# Autodesk Inventor assembly: SimplifiedLeg040x
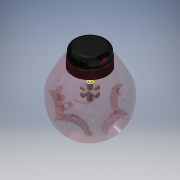
[picture p0: Inventor's stored thumbnail of the model, 180x180]
Saved by Autodesk Inventor 2018 (Build 220112000, 112)
## iProperties
Part Number: SimplifiedLeg040x
Material: Generisch
Document SubType Name: Assembly
Designer: Jochen Alt
Mass: 279.988 g
Surface Area: 1394.51 cm^2
Volume: 279.988 cm^3
Density: 1 g/cm^3
Author: Jochen Alt
## Documents named in this file (9)
- D:\Projects\Manfred\design\cad\simplified\SimplifiedLeg040x.iam
- D:\Projects\Manfred\design\cad\simplified\DrehAchse.ipt
- D:\Projects\Manfred\design\cad\simplified\SimplifiedFoot040x.ipt
- D:\Projects\Manfred\design\cad\simplified\SimplifiedThigh040x.ipt
- D:\Projects\Manfred\design\cad\simplified\SimplifiedHipJoint040x.ipt
- D:\Projects\Manfred\design\cad\simplified\SimplifiedHip040x.ipt
- D:\Projects\Manfred\design\cad\simplified\SimplifiedKnee040x.ipt
- D:\Projects\Manfred\design\cad\simplified\SimplifiedBody040x.ipt
- D:\Projects\Manfred\design\cad\Inventor\RPLidar A2.ipt
## Components (8 placed, 8 different names)
1. DrehAchse:1 — Passend:6, Passend:7, Passend:8, Passend:9, Passend:10, Passend:11, Passend:13, Passend:14, Winkel:1, Passend:15, Winkel:2
2. SimplifiedFoot040x:1 — Passend:6
3. SimplifiedThigh040x:1 — Passend:7, Passend:8
4. SimplifiedHipJoint040x:1 — Passend:9, Passend:10
5. SimplifiedHip040x:1 — Passend:11, Passend:15
6. SimplifiedKnee040x:1 — Passend:13, Passend:14, Winkel:1
7. SimplifiedBody040x:1 — Passend:16, Fluchtend:1
8. RPLidar A2:1 — Passend:16, Fluchtend:1, Winkel:2
## Relationships (13: Mate 10, Angle 2, Flush 1)
- Passend:6 [Mate]: DrehAchse:1 ↔ SimplifiedFoot040x:1
- Passend:7 [Mate]: DrehAchse:1 ↔ SimplifiedThigh040x:1
- Passend:8 [Mate]: DrehAchse:1 ↔ SimplifiedThigh040x:1
- Passend:9 [Mate]: DrehAchse:1 ↔ SimplifiedHipJoint040x:1
- Passend:10 [Mate]: DrehAchse:1 ↔ SimplifiedHipJoint040x:1
- Passend:11 [Mate]: DrehAchse:1 ↔ SimplifiedHip040x:1
- Passend:13 [Mate]: DrehAchse:1 ↔ SimplifiedKnee040x:1
- Passend:14 [Mate]: DrehAchse:1 ↔ SimplifiedKnee040x:1
- Winkel:1 [Angle] (180 deg): DrehAchse:1 ↔ SimplifiedKnee040x:1
- Passend:15 [Mate]: DrehAchse:1 ↔ SimplifiedHip040x:1
- Passend:16 [Mate]: SimplifiedBody040x:1 ↔ RPLidar A2:1
- Fluchtend:1 [Flush]: SimplifiedBody040x:1 ↔ RPLidar A2:1
- Winkel:2 [Angle] (0 deg): DrehAchse:1 ↔ RPLidar A2:1
